# Autodesk Inventor assembly: pistonMechanism-8-inV03
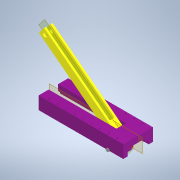
[picture p0: Inventor's stored thumbnail of the model, 180x180]
Saved by Autodesk Inventor 2020.2 (Build 242310000, 310)
## iProperties
Created: 2020-01-19
Part Number: pistonMechanism-8-inV03
Document SubType Name: Assembly
Designer: robst
Author: robst
## Documents named in this file (5)
- C:\git\CAD-Development\robSteele\2020BallTriggerMechanism\pistonMechanism-8-inV03.iam
- C:\git\CAD-Development\robSteele\2020BallTriggerMechanism\pistonHousingV03-8-in.ipt
- C:\git\CAD-Development\robSteele\2020BallTriggerMechanism\connectingRodV03-8-in.ipt
- C:\git\CAD-Development\robSteele\2020BallTriggerMechanism\pistonMechanism-8-inV03\Design Accelerator\Bolted Connection1.iam
- C:\git\CAD-Development\robSteele\2020BallTriggerMechanism\pistonFor-8-inV03.ipt
## Components (4 placed, 4 different names)
1. pistonHousingV03-8-in:1 — Mate:3, Mate:4
2. pistonFor-8-inV03:1 — Insert:1, Mate:1, Mate:2, Mate:3, Mate:4
3. connectingRodV03-8-in:1 — Insert:1
4. Bolted Connection:1 [sub-assembly] — Mate:1, Mate:2
## Relationships (5: Mate 4, Insert 1)
- Insert:1: pistonFor-8-inV03:1 ↔ connectingRodV03-8-in:1
- Mate:1: pistonFor-8-inV03:1 ↔ Bolted Connection:1
- Mate:2: pistonFor-8-inV03:1 ↔ Bolted Connection:1
- Mate:3: pistonHousingV03-8-in:1 ↔ pistonFor-8-inV03:1
- Mate:4: pistonHousingV03-8-in:1 ↔ pistonFor-8-inV03:1
